# Autodesk Inventor assembly: Ensamble2-1
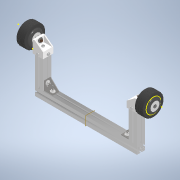
[picture p0: Inventor's stored thumbnail of the model, 180x180]
Saved by Autodesk Inventor 2021 (Build 250183000, 183)
## iProperties
Created: 2020-11-09
Part Number: Ensamble2-1
Document SubType Name: Assembly
Designer: juanm
Author: juanm
## Documents named in this file (20)
- C:\Users\juanm\OneDrive\Documentos\Inventor\NombreProyecto\Ensamble2-1.iam
- C:\Users\juanm\OneDrive\Documentos\Inventor\NombreProyecto\Horizontal.ipt
- C:\Users\juanm\OneDrive\Documentos\Inventor\NombreProyecto\Vertical.ipt
- C:\Users\juanm\OneDrive\Documentos\Inventor\NombreProyecto\Tornillo.ipt
- C:\Users\juanm\OneDrive\Documentos\Inventor\NombreProyecto\Sujetador2.ipt
- C:\Users\juanm\OneDrive\Documentos\Inventor\NombreProyecto\Tuerca para tornillo.ipt
- C:\Users\juanm\OneDrive\Documentos\Inventor\NombreProyecto\UnionLlantaOmega.ipt
- C:\Users\juanm\OneDrive\Documentos\Inventor\NombreProyecto\Tuerca.ipt
- C:\Users\juanm\OneDrive\Documentos\Inventor\NombreProyecto\Llanta.ipt
- C:\Users\juanm\OneDrive\Documentos\Inventor\NombreProyecto\Socket.ipt
- C:\Users\juanm\OneDrive\Documentos\Inventor\NombreProyecto\Rondana.ipt
- C:\Users\juanm\OneDrive\Documentos\Inventor\NombreProyecto\TuercaLlanta.ipt
- C:\Users\juanm\OneDrive\Documentos\Inventor\NombreProyecto\UnionLlantaOmega_MIR.ipt
- C:\Users\juanm\OneDrive\Documentos\Inventor\NombreProyecto\Tuerca_MIR.ipt
- C:\Users\juanm\OneDrive\Documentos\Inventor\NombreProyecto\Llanta_MIR.ipt
- C:\Users\juanm\OneDrive\Documentos\Inventor\NombreProyecto\Socket_MIR.ipt
- C:\Users\juanm\OneDrive\Documentos\Inventor\NombreProyecto\Rondana_MIR.ipt
- C:\Users\juanm\OneDrive\Documentos\Inventor\NombreProyecto\Rondana_MIR1.ipt
- C:\Users\juanm\OneDrive\Documentos\Inventor\NombreProyecto\TuercaLlanta_MIR.ipt
- C:\Users\juanm\OneDrive\Documentos\Inventor\NombreProyecto\Socket_MIR1.ipt
## Components (39 placed, 19 different names)
1. Horizontal:1 — Nivelación:1, Nivelación:2, Coincidencia:1, Coincidencia:5, Coincidencia:7, Nivelación:3, Coincidencia:8, Coincidencia:9, Coincidencia:11, Nivelación:4, Nivelación:5, Coincidencia:15, Coincidencia:16, Coincidencia:18, Coincidencia:20, Nivelación:6, Coincidencia:35, Coincidencia:36, Coincidencia:37, Coincidencia:38, Coincidencia:39
2. Vertical:2 — Nivelación:1, Nivelación:2, Coincidencia:1, Coincidencia:3, Coincidencia:4, Coincidencia:6, Coincidencia:10, Coincidencia:22, Coincidencia:23, Coincidencia:24, Coincidencia:25, Coincidencia:26, Coincidencia:27, Coincidencia:28, Coincidencia:29, Coincidencia:30, Coincidencia:31, Coincidencia:32, Coincidencia:33, Coincidencia:34, Nivelación:7, Nivelación:8
3. Tornillo:1 — Coincidencia:8, Coincidencia:9, Coincidencia:10, De rotación:2
4. Tornillo:2 — Coincidencia:3, Coincidencia:4, Coincidencia:5, De rotación:1
5. Sujetador2:1 — Coincidencia:6, Coincidencia:7, Nivelación:3
6. Tuerca para tornillo:1 — De rotación:2
7. Tuerca para tornillo:2 — De rotación:1
8. Vertical:3 — Coincidencia:11, Nivelación:4, Nivelación:5, Coincidencia:13, Coincidencia:14, Coincidencia:19, Coincidencia:21
9. Sujetador2:2 — Coincidencia:20, Coincidencia:21, Nivelación:6
10. Tornillo:3 — Coincidencia:13, Coincidencia:14, Coincidencia:15, De rotación:4
11. Tornillo:4 — Coincidencia:16, Coincidencia:18, Coincidencia:19, De rotación:3
12. Tuerca para tornillo:3 — De rotación:3
13. Tuerca para tornillo:4 — De rotación:4
14. UnionLlantaOmega:2 — Coincidencia:34, Nivelación:7, Nivelación:8, De rotación:5, De rotación:6, De rotación:7, De rotación:8, De rotación:9, De rotación:10
15. Tuerca:1 — Coincidencia:28, Coincidencia:29, Coincidencia:30
16. Tuerca:2 — Coincidencia:25, Coincidencia:26, Coincidencia:27
17. Tuerca:3 — Coincidencia:22, Coincidencia:23, Coincidencia:24
18. Tuerca:4 — Coincidencia:31, Coincidencia:32, Coincidencia:33
19. Llanta:1 — De rotación:5, De rotación:11, De rotación:18
20. Socket:1 — De rotación:9
21. Socket:2 — De rotación:7
22. Socket:3 — De rotación:8
23. Socket:4 — De rotación:6
24. Rondana:2 — De rotación:11
25. Socket:5 — De rotación:10
26. UnionLlantaOmega_MIR:1 — De rotación:12, De rotación:13, De rotación:14, De rotación:15, De rotación:17
27. Tuerca_MIR:1
28. Tuerca_MIR:2
29. Tuerca_MIR:3
30. Llanta_MIR:1 — De rotación:12, De rotación:16
31. Socket_MIR:1 — De rotación:13
32. Socket_MIR:2 — De rotación:14
33. Socket_MIR:3 — De rotación:15
34. Rondana_MIR:1 — De rotación:16
35. Socket_MIR:4 — De rotación:17
36. TuercaLlanta:1 — De rotación:18
37. Rondana_MIR1:1
38. TuercaLlanta_MIR:1
39. Socket_MIR1:1
## Relationships (62: Mate 36, RevoluteJoint 18, Flush 8)
- Nivelación:1 [Flush]: Horizontal:1 ↔ Vertical:2
- Nivelación:2 [Flush]: Horizontal:1 ↔ Vertical:2
- Coincidencia:1 [Mate]: Horizontal:1 ↔ Vertical:2
- Coincidencia:3 [Mate]: Vertical:2 ↔ Tornillo:2
- Coincidencia:4 [Mate] (2.3 mm): Vertical:2 ↔ Tornillo:2
- Coincidencia:5 [Mate] (24 mm): Horizontal:1 ↔ Tornillo:2
- Coincidencia:6 [Mate]: Vertical:2 ↔ Sujetador2:1
- Coincidencia:7 [Mate]: Horizontal:1 ↔ Sujetador2:1
- Nivelación:3 [Flush] (5 mm): Horizontal:1 ↔ Sujetador2:1
- Coincidencia:8 [Mate]: Horizontal:1 ↔ Tornillo:1
- Coincidencia:9 [Mate] (2.3 mm): Horizontal:1 ↔ Tornillo:1
- Coincidencia:10 [Mate] (24 mm): Vertical:2 ↔ Tornillo:1
- De rotación:1 [RevoluteJoint] (7 mm): Tornillo:2 ↔ Tuerca para tornillo:2
- De rotación:2 [RevoluteJoint] (-7 mm): Tornillo:1 ↔ Tuerca para tornillo:1
- Coincidencia:11 [Mate]: Horizontal:1 ↔ Vertical:3
- Nivelación:4 [Flush]: Horizontal:1 ↔ Vertical:3
- Nivelación:5 [Flush]: Horizontal:1 ↔ Vertical:3
- Coincidencia:13 [Mate]: Vertical:3 ↔ Tornillo:3
- Coincidencia:14 [Mate] (2.3 mm): Vertical:3 ↔ Tornillo:3
- Coincidencia:15 [Mate] (24 mm): Horizontal:1 ↔ Tornillo:3
- Coincidencia:16 [Mate]: Horizontal:1 ↔ Tornillo:4
- Coincidencia:18 [Mate] (2.3 mm): Horizontal:1 ↔ Tornillo:4
- Coincidencia:19 [Mate] (24 mm): Vertical:3 ↔ Tornillo:4
- Coincidencia:20 [Mate]: Horizontal:1 ↔ Sujetador2:2
- Coincidencia:21 [Mate]: Vertical:3 ↔ Sujetador2:2
- Nivelación:6 [Flush] (5 mm): Horizontal:1 ↔ Sujetador2:2
- De rotación:3 [RevoluteJoint] (-15 mm): Tornillo:4 ↔ Tuerca para tornillo:3
- De rotación:4 [RevoluteJoint] (15 mm): Tornillo:3 ↔ Tuerca para tornillo:4
- Coincidencia:22 [Mate] (-27.5 mm): Vertical:2 ↔ Tuerca:3
- Coincidencia:23 [Mate]: Vertical:2 ↔ Tuerca:3
- Coincidencia:24 [Mate] (3 mm): Vertical:2 ↔ Tuerca:3
- Coincidencia:25 [Mate] (-27.5 mm): Vertical:2 ↔ Tuerca:2
- Coincidencia:26 [Mate]: Vertical:2 ↔ Tuerca:2
- Coincidencia:27 [Mate] (3.1 mm): Vertical:2 ↔ Tuerca:2
- Coincidencia:28 [Mate] (-27.5 mm): Vertical:2 ↔ Tuerca:1
- Coincidencia:29 [Mate] (3.1 mm): Vertical:2 ↔ Tuerca:1
- Coincidencia:30 [Mate]: Vertical:2 ↔ Tuerca:1
- Coincidencia:31 [Mate] (-27.5 mm): Vertical:2 ↔ Tuerca:4
- Coincidencia:32 [Mate] (3.1 mm): Vertical:2 ↔ Tuerca:4
- Coincidencia:33 [Mate]: Vertical:2 ↔ Tuerca:4
- Coincidencia:34 [Mate]: Vertical:2 ↔ UnionLlantaOmega:2
- Nivelación:7 [Flush] (-5 mm): Vertical:2 ↔ UnionLlantaOmega:2
- Nivelación:8 [Flush] (-5 mm): Vertical:2 ↔ UnionLlantaOmega:2
- De rotación:5 [RevoluteJoint] (-10 mm): UnionLlantaOmega:2 ↔ Llanta:1
- De rotación:6 [RevoluteJoint] (16 mm): UnionLlantaOmega:2 ↔ Socket:4
- De rotación:7 [RevoluteJoint] (16 mm): UnionLlantaOmega:2 ↔ Socket:2
- De rotación:8 [RevoluteJoint] (16 mm): UnionLlantaOmega:2 ↔ Socket:3
- De rotación:9 [RevoluteJoint] (16 mm): UnionLlantaOmega:2 ↔ Socket:1
- De rotación:10 [RevoluteJoint] (16 mm): UnionLlantaOmega:2 ↔ Socket:5
- De rotación:11 [RevoluteJoint] (-22.5 mm): Llanta:1 ↔ Rondana:2
- Coincidencia:35 [Mate]: Horizontal:1
- Coincidencia:36 [Mate]: Horizontal:1
- Coincidencia:37 [Mate]: Horizontal:1
- Coincidencia:38 [Mate]: Horizontal:1
- Coincidencia:39 [Mate]: Horizontal:1
- De rotación:12 [RevoluteJoint] (10 mm): UnionLlantaOmega_MIR:1 ↔ Llanta_MIR:1
- De rotación:13 [RevoluteJoint] (-16 mm): UnionLlantaOmega_MIR:1 ↔ Socket_MIR:1
- De rotación:14 [RevoluteJoint] (-16 mm): UnionLlantaOmega_MIR:1 ↔ Socket_MIR:2
- De rotación:15 [RevoluteJoint] (-16 mm): UnionLlantaOmega_MIR:1 ↔ Socket_MIR:3
- De rotación:16 [RevoluteJoint] (22.5 mm): Llanta_MIR:1 ↔ Rondana_MIR:1
- De rotación:17 [RevoluteJoint] (-16 mm): UnionLlantaOmega_MIR:1 ↔ Socket_MIR:4
- De rotación:18 [RevoluteJoint] (-5 mm): Llanta:1 ↔ TuercaLlanta:1
